# Autodesk Inventor assembly: POM_T5_03
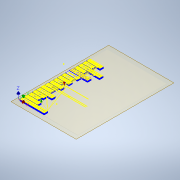
[picture p0: Inventor's stored thumbnail of the model, 180x180]
Saved by Autodesk Inventor 2020 (Build 240168000, 168)
## iProperties
Created: 2021-08-27
Part Number: POM_T5_03
Document SubType Name: Assembly
Designer: Masato
Author: Masato
## Documents named in this file (19)
- C:\Users\L20C1118 森　圭汰\Documents\211019_open\OpenPlatform_ver3_0\cam\POM_T5_03.iam
- C:\Users\L20C1118 森　圭汰\Documents\211019_open\OpenPlatform_ver3_0\cam\Disposable_Board.ipt
- C:\Users\L20C1118 森　圭汰\Documents\211022_open\OpenPlatform_ver3_0\JIG\BackLink_diagonal_jig.ipt
- C:\Users\L20C1118 森　圭汰\Documents\211022_open\OpenPlatform_ver3_0\JIG\Camera_side_frame_jig.ipt
- C:\Users\L20C1118 森　圭汰\Documents\211022_open\OpenPlatform_ver3_0\JIG\Foot_root_block_jig.ipt
- C:\Users\L20C1118 森　圭汰\Documents\211022_open\OpenPlatform_ver3_0\JIG\ForeArm_diagonal_jig_01.ipt
- C:\Users\L20C1118 森　圭汰\Documents\211022_open\OpenPlatform_ver3_0\JIG\ForeArm_diagonal_jig_02.ipt
- C:\Users\L20C1118 森　圭汰\Documents\211022_open\OpenPlatform_ver3_0\JIG\ForeArm_diagonal_jig_03.ipt
- C:\Users\L20C1118 森　圭汰\Documents\211022_open\OpenPlatform_ver3_0\JIG\FrontLink_diagonal_jig.ipt
- C:\Users\L20C1118 森　圭汰\Documents\211022_open\OpenPlatform_ver3_0\JIG\Head_diagonal_jig.ipt
- C:\Users\L20C1118 森　圭汰\Documents\211022_open\OpenPlatform_ver3_0\JIG\Head_horn_frame_jig.ipt
- C:\Users\L20C1118 森　圭汰\Documents\211022_open\OpenPlatform_ver3_0\JIG\Leg_joint_yaw_frame_jig.ipt
- C:\Users\L20C1118 森　圭汰\Documents\211022_open\OpenPlatform_ver3_0\JIG\Shoulder_horn_frame_jig.ipt
- C:\Users\L20C1118 森　圭汰\Documents\211022_open\OpenPlatform_ver3_0\JIG\Trunk_ampit_frame_jig_01.ipt
- C:\Users\L20C1118 森　圭汰\Documents\211022_open\OpenPlatform_ver3_0\JIG\Trunk_ampit_frame_jig_02.ipt
- C:\Users\L20C1118 森　圭汰\Documents\211022_open\OpenPlatform_ver3_0\JIG\Trunk_chest_back_forth_frame_jig_01.ipt
- C:\Users\L20C1118 森　圭汰\Documents\211022_open\OpenPlatform_ver3_0\JIG\Trunk_chest_back_forth_frame_jig_02.ipt
- C:\Users\L20C1118 森　圭汰\Documents\211022_open\OpenPlatform_ver3_0\JIG\Trunk_lower_flank_frame_jig.ipt
- C:\Users\L20C1118 森　圭汰\Documents\211022_open\OpenPlatform_ver3_0\JIG\UpperArm_diagonal_jig.ipt
## Components (18 placed, 18 different names)
1. Disposable_Board:1 — メイト:2, メイト:1, フラッシュ:1, フラッシュ:2, フラッシュ:3, フラッシュ:4
2. BackLink_diagonal_jig:1 — メイト:4, フラッシュ:14, メイト:35, メイト:36
3. Camera_side_frame_jig:1 — メイト:5, フラッシュ:18, メイト:32, メイト:33
4. Foot_root_block_jig:1 — メイト:6, フラッシュ:11, メイト:30, メイト:31
5. ForeArm_diagonal_jig_01:1 — メイト:7, フラッシュ:19, メイト:23, メイト:24
6. ForeArm_diagonal_jig_02:1 — メイト:8, フラッシュ:15, メイト:28, メイト:29
7. ForeArm_diagonal_jig_03:1 — メイト:9, フラッシュ:20, メイト:26, メイト:27
8. FrontLink_diagonal_jig:1 — メイト:10, フラッシュ:17, メイト:24, メイト:25
9. Head_diagonal_jig:1 — メイト:14, フラッシュ:8, メイト:22, メイト:23
10. Head_horn_frame_jig:1 — メイト:13, フラッシュ:10, メイト:33, メイト:34
11. Leg_joint_yaw_frame_jig:1 — メイト:15, フラッシュ:7, メイト:25, メイト:26
12. Shoulder_horn_frame_jig:1 — メイト:12, フラッシュ:13, メイト:29, メイト:30
13. Trunk_ampit_frame_jig_01:1 — メイト:11, フラッシュ:16, メイト:21, メイト:22
14. Trunk_ampit_frame_jig_02:1 — メイト:16, フラッシュ:9, メイト:36
15. Trunk_chest_back_forth_frame_jig_01:1 — メイト:17, フラッシュ:3, フラッシュ:4, フラッシュ:5, フラッシュ:6, フラッシュ:7, フラッシュ:8, フラッシュ:9, フラッシュ:10, フラッシュ:11, フラッシュ:12, フラッシュ:13, フラッシュ:14, フラッシュ:15, フラッシュ:16, フラッシュ:17, フラッシュ:18, フラッシュ:19, フラッシュ:20, メイト:21
16. Trunk_chest_back_forth_frame_jig_02:1 — メイト:18, フラッシュ:5, メイト:27, メイト:28
17. Trunk_lower_flank_frame_jig:1 — メイト:19, フラッシュ:12, メイト:34, メイト:35
18. UpperArm_diagonal_jig:1 — メイト:20, フラッシュ:6, メイト:31, メイト:32
## Relationships (55: Mate 35, Flush 20)
- メイト:2 [Mate]: Disposable_Board:1
- メイト:1 [Mate]: Disposable_Board:1
- フラッシュ:1 [Flush]: Disposable_Board:1
- フラッシュ:2 [Flush]: Disposable_Board:1
- メイト:4 [Mate]: BackLink_diagonal_jig:1
- メイト:5 [Mate]: Camera_side_frame_jig:1
- メイト:6 [Mate]: Foot_root_block_jig:1
- メイト:7 [Mate]: ForeArm_diagonal_jig_01:1
- メイト:8 [Mate]: ForeArm_diagonal_jig_02:1
- メイト:9 [Mate]: ForeArm_diagonal_jig_03:1
- メイト:10 [Mate]: FrontLink_diagonal_jig:1
- メイト:11 [Mate]: Trunk_ampit_frame_jig_01:1
- メイト:12 [Mate]: Shoulder_horn_frame_jig:1
- メイト:13 [Mate]: Head_horn_frame_jig:1
- メイト:14 [Mate]: Head_diagonal_jig:1
- メイト:15 [Mate]: Leg_joint_yaw_frame_jig:1
- メイト:16 [Mate]: Trunk_ampit_frame_jig_02:1
- メイト:17 [Mate]: Trunk_chest_back_forth_frame_jig_01:1
- メイト:18 [Mate]: Trunk_chest_back_forth_frame_jig_02:1
- メイト:19 [Mate]: Trunk_lower_flank_frame_jig:1
- メイト:20 [Mate]: UpperArm_diagonal_jig:1
- フラッシュ:3 [Flush] (3 mm): Disposable_Board:1 ↔ Trunk_chest_back_forth_frame_jig_01:1
- フラッシュ:4 [Flush] (3 mm): Disposable_Board:1 ↔ Trunk_chest_back_forth_frame_jig_01:1
- フラッシュ:5 [Flush]: Trunk_chest_back_forth_frame_jig_01:1 ↔ Trunk_chest_back_forth_frame_jig_02:1
- フラッシュ:6 [Flush]: Trunk_chest_back_forth_frame_jig_01:1 ↔ UpperArm_diagonal_jig:1
- フラッシュ:7 [Flush]: Leg_joint_yaw_frame_jig:1 ↔ Trunk_chest_back_forth_frame_jig_01:1
- フラッシュ:8 [Flush]: Head_diagonal_jig:1 ↔ Trunk_chest_back_forth_frame_jig_01:1
- フラッシュ:9 [Flush]: Trunk_ampit_frame_jig_02:1 ↔ Trunk_chest_back_forth_frame_jig_01:1
- フラッシュ:10 [Flush]: Head_horn_frame_jig:1 ↔ Trunk_chest_back_forth_frame_jig_01:1
- フラッシュ:11 [Flush]: Foot_root_block_jig:1 ↔ Trunk_chest_back_forth_frame_jig_01:1
- フラッシュ:12 [Flush]: Trunk_chest_back_forth_frame_jig_01:1 ↔ Trunk_lower_flank_frame_jig:1
- フラッシュ:13 [Flush]: Shoulder_horn_frame_jig:1 ↔ Trunk_chest_back_forth_frame_jig_01:1
- フラッシュ:14 [Flush]: BackLink_diagonal_jig:1 ↔ Trunk_chest_back_forth_frame_jig_01:1
- フラッシュ:15 [Flush]: ForeArm_diagonal_jig_02:1 ↔ Trunk_chest_back_forth_frame_jig_01:1
- フラッシュ:16 [Flush]: Trunk_ampit_frame_jig_01:1 ↔ Trunk_chest_back_forth_frame_jig_01:1
- フラッシュ:17 [Flush]: FrontLink_diagonal_jig:1 ↔ Trunk_chest_back_forth_frame_jig_01:1
- フラッシュ:18 [Flush]: Camera_side_frame_jig:1 ↔ Trunk_chest_back_forth_frame_jig_01:1
- フラッシュ:19 [Flush]: ForeArm_diagonal_jig_01:1 ↔ Trunk_chest_back_forth_frame_jig_01:1
- フラッシュ:20 [Flush]: ForeArm_diagonal_jig_03:1 ↔ Trunk_chest_back_forth_frame_jig_01:1
- メイト:21 [Mate] (3 mm): Trunk_ampit_frame_jig_01:1 ↔ Trunk_chest_back_forth_frame_jig_01:1
- メイト:22 [Mate] (3 mm): Head_diagonal_jig:1 ↔ Trunk_ampit_frame_jig_01:1
- メイト:23 [Mate] (3 mm): ForeArm_diagonal_jig_01:1 ↔ Head_diagonal_jig:1
- メイト:24 [Mate] (3 mm): ForeArm_diagonal_jig_01:1 ↔ FrontLink_diagonal_jig:1
- メイト:25 [Mate] (3 mm): FrontLink_diagonal_jig:1 ↔ Leg_joint_yaw_frame_jig:1
- メイト:26 [Mate] (3 mm): ForeArm_diagonal_jig_03:1 ↔ Leg_joint_yaw_frame_jig:1
- メイト:27 [Mate] (3 mm): ForeArm_diagonal_jig_03:1 ↔ Trunk_chest_back_forth_frame_jig_02:1
- メイト:28 [Mate] (3 mm): ForeArm_diagonal_jig_02:1 ↔ Trunk_chest_back_forth_frame_jig_02:1
- メイト:29 [Mate] (3 mm): ForeArm_diagonal_jig_02:1 ↔ Shoulder_horn_frame_jig:1
- メイト:30 [Mate] (3 mm): Foot_root_block_jig:1 ↔ Shoulder_horn_frame_jig:1
- メイト:31 [Mate] (3 mm): Foot_root_block_jig:1 ↔ UpperArm_diagonal_jig:1
- メイト:32 [Mate] (3 mm): Camera_side_frame_jig:1 ↔ UpperArm_diagonal_jig:1
- メイト:33 [Mate] (3 mm): Camera_side_frame_jig:1 ↔ Head_horn_frame_jig:1
- メイト:34 [Mate] (3 mm): Head_horn_frame_jig:1 ↔ Trunk_lower_flank_frame_jig:1
- メイト:35 [Mate] (3 mm): BackLink_diagonal_jig:1 ↔ Trunk_lower_flank_frame_jig:1
- メイト:36 [Mate] (3 mm): BackLink_diagonal_jig:1 ↔ Trunk_ampit_frame_jig_02:1
